# Autodesk Inventor assembly: aileron_assembly
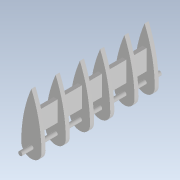
[picture p0: Inventor's stored thumbnail of the model, 180x180]
Saved by Autodesk Inventor 2020 (Build 240168000, 168)
## iProperties
Created: 2020-09-10
Part Number: aileron_assembly
Document SubType Name: Assembly
Designer: Admin
Author: Admin
## Documents named in this file (4)
- C:\PFE\Project_github\YFA-Project_python_interface\3D models\aileron_assembly.iam
- C:\PFE\Project_github\YFA-Project_python_interface\3D models\aileron_arriere.ipt
- C:\PFE\Project_github\YFA-Project_python_interface\3D models\aileron_traverse.ipt
- C:\PFE\Project_github\YFA-Project_python_interface\3D models\axe_aileron.ipt
## Components (8 placed, 3 different names)
1. aileron_arriere:1 — Flush:1, Mate:8, Mate:9, Flush:3, Flush:4, Mate:16
2. aileron_arriere:2 — Flush:1, Mate:1, Mate:7, Mate:8, Mate:10
3. aileron_arriere:3 — Mate:1, Flush:2, Mate:6, Mate:7, Mate:11, Mate:15
4. aileron_arriere:4 — Flush:2, Mate:2, Mate:5, Mate:6, Mate:13
5. aileron_arriere:5 — Mate:2, Mate:3, Mate:4, Mate:5, Mate:14
6. aileron_arriere:6 — Mate:3, Mate:4, Mate:12
7. aileron_traverse:1 — Mate:9, Mate:10, Mate:11, Mate:12, Mate:13, Mate:14, Flush:3, Mate:15
8. axe_aileron:1 — Flush:4, Mate:16
## Relationships (20: Mate 16, Flush 4)
- Flush:1 (10 mm): aileron_arriere:1 ↔ aileron_arriere:2
- Mate:1 (10 mm): aileron_arriere:2 ↔ aileron_arriere:3
- Flush:2 (10 mm): aileron_arriere:3 ↔ aileron_arriere:4
- Mate:2 (10 mm): aileron_arriere:4 ↔ aileron_arriere:5
- Mate:3 (10 mm): aileron_arriere:5 ↔ aileron_arriere:6
- Mate:4: aileron_arriere:5 ↔ aileron_arriere:6
- Mate:5: aileron_arriere:4 ↔ aileron_arriere:5
- Mate:6: aileron_arriere:3 ↔ aileron_arriere:4
- Mate:7: aileron_arriere:2 ↔ aileron_arriere:3
- Mate:8: aileron_arriere:1 ↔ aileron_arriere:2
- Mate:9: aileron_arriere:1 ↔ aileron_traverse:1
- Mate:10: aileron_arriere:2 ↔ aileron_traverse:1
- Mate:11: aileron_arriere:3 ↔ aileron_traverse:1
- Mate:12: aileron_arriere:6 ↔ aileron_traverse:1
- Mate:13: aileron_arriere:4 ↔ aileron_traverse:1
- Mate:14: aileron_arriere:5 ↔ aileron_traverse:1
- Flush:3: aileron_arriere:1 ↔ aileron_traverse:1
- Mate:15: aileron_arriere:3 ↔ aileron_traverse:1
- Flush:4 (5.5 mm): aileron_arriere:1 ↔ axe_aileron:1
- Mate:16: aileron_arriere:1 ↔ axe_aileron:1
